# Autodesk Inventor assembly: Front Left Foot
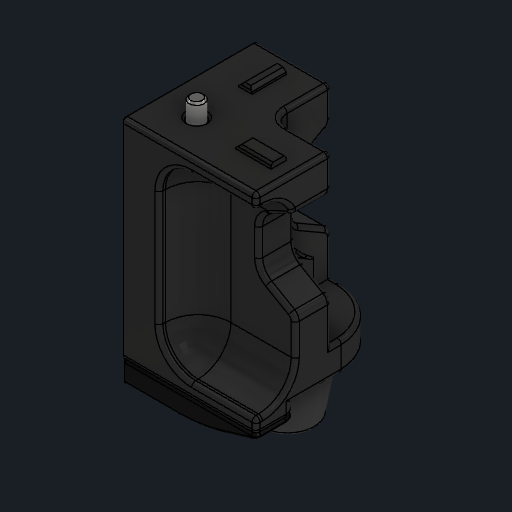
[picture p0: Inventor's stored thumbnail of the model, 512x512]
Saved by Autodesk Inventor 2026.1 (Build 301233020, 233B)
## iProperties
Created: 2025-05-09
Part Number: Front Left Foot
Document SubType Name: Assembly
Designer: AdminForWorker
Title: Front Left Foot
Author: AdminForWorker
## Documents named in this file (8)
- C:\Users\JoshuaEah\Documents\GitHub\Voron-0\CAD\Master Assembly\Skirt\Feet\Front Left Foot.iam
- C:\Users\JoshuaEah\Documents\GitHub\Voron-0\CAD\Master Assembly\Hardware\M3 Threaded Insert.ipt
- C:\Users\JoshuaEah\Documents\GitHub\Voron-0\CAD\Master Assembly\Hardware\M2x10 Self Tapper.ipt
- C:\Users\JoshuaEah\Documents\GitHub\Voron-0\CAD\Master Assembly\Hardware\M3x40 BHCS.ipt
- C:\Users\JoshuaEah\Documents\GitHub\Voron-0\CAD\Master Assembly\Hardware\M3x10 BHCS.ipt
- C:\Users\JoshuaEah\Documents\GitHub\Voron-0\CAD\Master Assembly\Skirt\Feet\Rubber Foot.ipt
- C:\Users\JoshuaEah\Documents\GitHub\Voron-0\CAD\Master Assembly\Skirt\Feet\Front Left Foot (1).ipt
- C:\Users\JoshuaEah\Documents\GitHub\Voron-0\CAD\Master Assembly\Skirt\Feet\Foot Accent.ipt
## Components (8 placed, 7 different names)
1. M3 Threaded Insert (1) (2):1
2. M2x10 Self Tapper:1
3. M2x10 Self Tapper:2
4. M3x40 BHCS:1
5. M3x10 BHCS:1
6. Rubber Foot:1
7. Front Left Foot (1):1
8. Foot Accent (2):1
## Relationships (2: Insert 2)
- [Insert]: M2x10 Self Tapper:1 ↔ Foot Accent (2):1
- [Insert]: M2x10 Self Tapper:2 ↔ Foot Accent (2):1
